# Autodesk Inventor assembly: Tablero
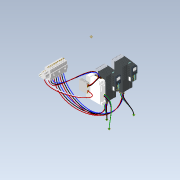
[picture p0: Inventor's stored thumbnail of the model, 180x180]
Saved by Autodesk Inventor 2021 (Build 250183000, 183)
## iProperties
Created: 2021-08-19
Part Number: Tablero
Document SubType Name: Assembly
Designer: Andrés Holguín
Author: Andrés Holguín
## Documents named in this file (10)
- C:\Users\andre\Documents\GitHub\Dis.-Mecatronico-E6\inventor proyecto\Tablero\Tablero.iam
- C:\Users\andre\Documents\GitHub\Dis.-Mecatronico-E6\inventor proyecto\Tablero\Variador\_G120_3D_bc0ba93eda2faaeaa13b0d790d7aac92.iam
- C:\Users\andre\Documents\GitHub\Dis.-Mecatronico-E6\inventor proyecto\Tablero\DriveActuador\AIS2021\8133356 CMMT-AS-C7-11A-P3-EP-S1.iam
- C:\Users\andre\Documents\GitHub\Dis.-Mecatronico-E6\inventor proyecto\Tablero\DriveActuador\2247681 CACN-3A-1-5.ipt
- C:\Users\andre\Documents\GitHub\Dis.-Mecatronico-E6\inventor proyecto\Tablero\Tablero.Harness1.iam
- C:\Users\andre\Documents\GitHub\Dis.-Mecatronico-E6\inventor proyecto\Tablero\Extra\pin.ipt
- C:\Users\andre\Documents\GitHub\Dis.-Mecatronico-E6\inventor proyecto\Tablero\Riel DIN\Riel DIN.ipt
- C:\Users\andre\Documents\GitHub\Dis.-Mecatronico-E6\inventor proyecto\Tablero\Interruptores\3p50.ipt
- C:\Users\andre\Documents\GitHub\Dis.-Mecatronico-E6\inventor proyecto\Tablero\Interruptores\3p30.ipt
- C:\Users\andre\Documents\GitHub\Dis.-Mecatronico-E6\inventor proyecto\Tablero\Interruptores\2p8\a9n18344.iam
## Components (14 placed, 9 different names)
1. _G120_3D_bc0ba93eda2faaeaa13b0d790d7aac92:1 [sub-assembly]
2. _G120_3D_bc0ba93eda2faaeaa13b0d790d7aac92:2 [sub-assembly]
3. 2247681 CACN-3A-1-5:1
4. 8133356 CMMT-AS-C7-11A-P3-EP-S1:1 [sub-assembly]
5. Harness1 [sub-assembly]
6. pin:1
7. pin:2
8. pin:3
9. Riel DIN:1 — Mate:1
10. pin:4
11. 3p50:1 — Rigid:1, Mate:1, Rigid:2
12. 3p50:2 — Rigid:1
13. 3p30:1 — Rigid:2, Rigid:3
14. a9n18344:1 [sub-assembly] — Rigid:3
## Relationships (4: WeldJoint 3, Mate 1)
- Rigid:1 [WeldJoint]: 3p50:1 ↔ 3p50:2
- Mate:1: Riel DIN:1 ↔ 3p50:1
- Rigid:2 [WeldJoint]: 3p50:1 ↔ 3p30:1
- Rigid:3 [WeldJoint]: 3p30:1 ↔ a9n18344:1
